# Autodesk Inventor assembly: mic
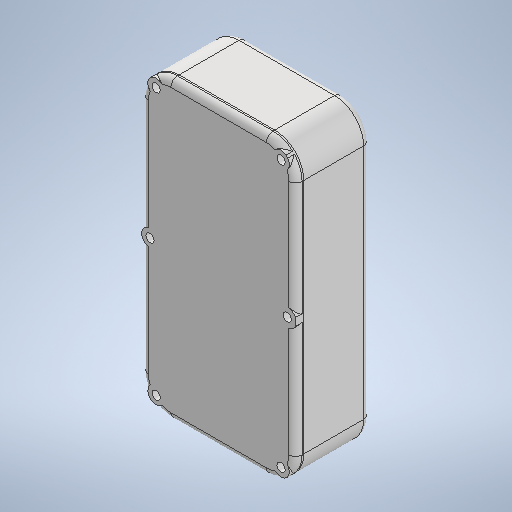
[picture p0: Inventor's stored thumbnail of the model, 512x512]
Saved by Autodesk Inventor 2025.2 (Build 292293000, 293)
## iProperties
Created: 2025-04-18
Part Number: mic
Document SubType Name: Assembly
Designer: tdeboutte
Author: tdeboutte
## Documents named in this file (3)
- C:\Users\tdeboutte\Documents\Projects\bluesmobile\bluesmobile-cad\mic.iam
- C:\Users\tdeboutte\Documents\Projects\bluesmobile\bluesmobile-cad\mic-base.ipt
- C:\Users\tdeboutte\Documents\Projects\bluesmobile\bluesmobile-cad\mic-front.ipt
## Components (2 placed, 2 different names)
1. mic-base:1 — Flush:1, Flush:2, Flush:3
2. mic-front:1 — Flush:1, Flush:2, Flush:3
## Relationships (3: Flush 3)
- Flush:1: mic-base:1 ↔ mic-front:1
- Flush:2: mic-base:1 ↔ mic-front:1
- Flush:3: mic-base:1 ↔ mic-front:1
